# Autodesk Inventor assembly: клешня сбора
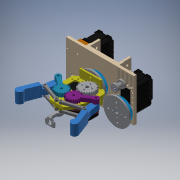
[picture p0: Inventor's stored thumbnail of the model, 180x180]
Saved by Autodesk Inventor 2019 (Build 230136000, 136)
## iProperties
Created: 2019-08-15
Part Number: клешня сбора
Material: Типовые
Document SubType Name: Assembly
Designer: Петров Иван
Mass: 338.18 g
Surface Area: 1360.82 cm^2
Volume: 291.895 cm^3
Density: 1.15857 g/cm^3
Author: Петров Иван
## Documents named in this file (10)
- E:\IVAN\Kvantoriada20192\optimal_gripper\hardware\КВ33.044.100 - Захват.iam
- E:\IVAN\Kvantoriada20192\optimal_gripper\hardware\КВ33.044.101 - Опора захвата.ipt
- E:\IVAN\Kvantoriada20192\optimal_gripper\hardware\Стандартные изделия\Сервомотор Dynamixel AX-12A\AX-12.iam
- E:\IVAN\Kvantoriada20192\optimal_gripper\hardware\Стандартные изделия\Проставка 4 мм.ipt
- E:\IVAN\Kvantoriada20192\optimal_gripper\hardware\Стандартные изделия\Шкив большой Makeblock.ipt
- E:\IVAN\Kvantoriada20192\optimal_gripper\hardware\Стандартные изделия\Боковина шкива уменьшанная.ipt
- E:\IVAN\Kvantoriada20192\optimal_gripper\hardware\Стандартные изделия\Шкив большой сборка.iam
- E:\IVAN\Kvantoriada20192\optimal_gripper\hardware\КВ33.044.200 - Сборка зажима.iam
- E:\IVAN\Kvantoriada20192\optimal_gripper\hardware\Стандартные изделия\Шкив плоский Makeblock сборка.iam
- E:\IVAN\Kvantoriada20192\optimal_gripper\hardware\КВ33.044.900 - Клапан присоски впускной.iam
## Components (10 placed, 9 different names)
1. КВ33.044.101 - Опора захвата:1 — Совмещение:17, Совмещение:18, Совмещение:25, Касательность:1, Касательность:2, Совмещение:28, Совмещение:29, Совмещение:30, Совмещение:31, Совмещение:32, Совмещение:33
2. AX-12:1 [sub-assembly] — Совмещение:31, Совмещение:32, Совмещение:33, Совмещение:34, Совмещение:35
3. Проставка 4 мм:1 — Совмещение:6, Совмещение:7, Совмещение:8, Совмещение:34
4. Шкив большой Makeblock:1 — Совмещение:6, Совмещение:7, Совмещение:8, Совмещение:14, Совмещение:15, Совмещение:16, Направление навивки:1
5. Боковина шкива уменьшанная:1 — Совмещение:14, Совмещение:15, Совмещение:16, Совмещение:35, Направление навивки:2
6. Шкив большой сборка:1 [sub-assembly] — Совмещение:17, Совмещение:18, Направление навивки:1, Совмещение:19, Совмещение:20, Совмещение:21
7. Боковина шкива уменьшанная:2 — Совмещение:19, Совмещение:20, Совмещение:21, Совмещение:22, Совмещение:23, Совмещение:24
8. КВ33.044.200 - Сборка зажима:1 [sub-assembly] — Совмещение:22, Совмещение:23, Совмещение:24
9. Шкив плоский Makeblock сборка:1 [sub-assembly] — Совмещение:25, Касательность:1, Касательность:2, Направление навивки:2
10. КВ33.044.900 - Клапан присоски впускной:1 [sub-assembly] — Совмещение:28, Совмещение:29, Совмещение:30
## Relationships (27: Mate 23, RelateRotation 2, Tangent 2)
- Совмещение:6 [Mate]: Проставка 4 мм:1 ↔ Шкив большой Makeblock:1
- Совмещение:7 [Mate]: Проставка 4 мм:1 ↔ Шкив большой Makeblock:1
- Совмещение:8 [Mate]: Проставка 4 мм:1 ↔ Шкив большой Makeblock:1
- Совмещение:14 [Mate]: Шкив большой Makeblock:1 ↔ Боковина шкива уменьшанная:1
- Совмещение:15 [Mate]: Шкив большой Makeblock:1 ↔ Боковина шкива уменьшанная:1
- Совмещение:16 [Mate]: Шкив большой Makeblock:1 ↔ Боковина шкива уменьшанная:1
- Совмещение:17 [Mate] (4.24 mm): КВ33.044.101 - Опора захвата:1 ↔ Шкив большой сборка:1
- Совмещение:18 [Mate]: КВ33.044.101 - Опора захвата:1 ↔ Шкив большой сборка:1
- Направление навивки:1 [RelateRotation] (1 ul): Шкив большой Makeblock:1 ↔ Шкив большой сборка:1
- Совмещение:19 [Mate]: Шкив большой сборка:1 ↔ Боковина шкива уменьшанная:2
- Совмещение:20 [Mate]: Шкив большой сборка:1 ↔ Боковина шкива уменьшанная:2
- Совмещение:21 [Mate]: Шкив большой сборка:1 ↔ Боковина шкива уменьшанная:2
- Совмещение:22 [Mate]: Боковина шкива уменьшанная:2 ↔ КВ33.044.200 - Сборка зажима:1
- Совмещение:23 [Mate]: Боковина шкива уменьшанная:2 ↔ КВ33.044.200 - Сборка зажима:1
- Совмещение:24 [Mate]: Боковина шкива уменьшанная:2 ↔ КВ33.044.200 - Сборка зажима:1
- Совмещение:25 [Mate]: КВ33.044.101 - Опора захвата:1 ↔ Шкив плоский Makeblock сборка:1
- Касательность:1 [Tangent]: КВ33.044.101 - Опора захвата:1 ↔ Шкив плоский Makeblock сборка:1
- Касательность:2 [Tangent]: КВ33.044.101 - Опора захвата:1 ↔ Шкив плоский Makeblock сборка:1
- Совмещение:28 [Mate]: КВ33.044.101 - Опора захвата:1 ↔ КВ33.044.900 - Клапан присоски впускной:1
- Совмещение:29 [Mate]: КВ33.044.101 - Опора захвата:1 ↔ КВ33.044.900 - Клапан присоски впускной:1
- Совмещение:30 [Mate]: КВ33.044.101 - Опора захвата:1 ↔ КВ33.044.900 - Клапан присоски впускной:1
- Совмещение:31 [Mate]: КВ33.044.101 - Опора захвата:1 ↔ AX-12:1
- Совмещение:32 [Mate]: КВ33.044.101 - Опора захвата:1 ↔ AX-12:1
- Совмещение:33 [Mate]: КВ33.044.101 - Опора захвата:1 ↔ AX-12:1
- Совмещение:34 [Mate]: AX-12:1 ↔ Проставка 4 мм:1
- Совмещение:35 [Mate]: AX-12:1 ↔ Боковина шкива уменьшанная:1
- Направление навивки:2 [RelateRotation] (0.2 ul): Боковина шкива уменьшанная:1 ↔ Шкив плоский Makeblock сборка:1
